# Autodesk Inventor assembly: 20263829
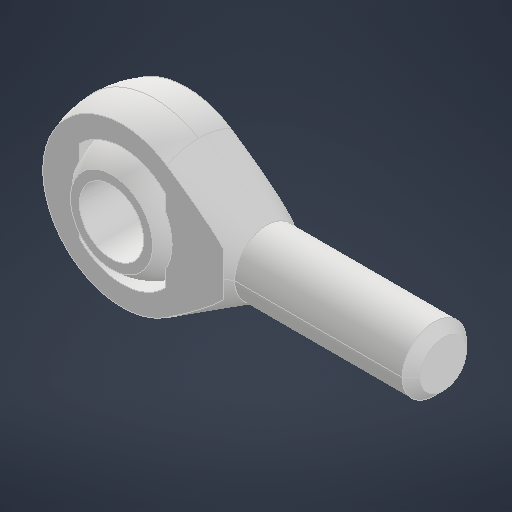
[picture p0: Inventor's stored thumbnail of the model, 512x512]
Saved by Autodesk Inventor 2026.1 (Build 301233000, 233)
## iProperties
Company: TraceParts S.A.
Created: 2026-06-12
Part Number: 20263829
Checked By: TraceParts S.A.
Catalog Web Link: www.traceparts.com
Document SubType Name: Assembly
Designer: TraceParts
Sending System: TraceParts v2
Major Version: 6.0
Minor Version: 0.0
Format Version: 0.0
Product Id: TraceParts v2
REFERENCE: 20263829
SUPPLIER: Essentra Components
DESIGN: Heavy Duty Rod End 12.0 54.0 M12 Steel
TraceParts.PartNumber: 90-24072024-043323
TraceParts.PartTitle: Heavy Duty Rod End 12.0 54.0 M12 Steel
TraceParts.InstanceId: 90-24072024-04332395OX6XW0EVGZUOK7QRY6KRUYN
TRACEPARTS: TRACEPARTS
TraceParts.PartLanguage: en
TraceParts.PartVersion: 1.0.1
Author: TraceParts
## Documents named in this file (4)
- C:\Users\share\OneDrive\Documents\Personal Projects\GOGO Kart\CAD\GOGO_KART_FSAE\Suspension\Suspension Parts\Front Upper Arm\Rod End CAD Files\185237224-9-20263829\20263829.iam
- C:\Users\share\OneDrive\Documents\Personal Projects\GOGO Kart\CAD\GOGO_KART_FSAE\Suspension\Suspension Parts\Front Upper Arm\Rod End CAD Files\185237224-9-20263829\20263829_01.ipt
- C:\Users\share\OneDrive\Documents\Personal Projects\GOGO Kart\CAD\GOGO_KART_FSAE\Suspension\Suspension Parts\Front Upper Arm\Rod End CAD Files\185237224-9-20263829\20263829_02.ipt
- C:\Users\share\OneDrive\Documents\Personal Projects\GOGO Kart\CAD\GOGO_KART_FSAE\Suspension\Suspension Parts\Front Upper Arm\Rod End CAD Files\185237224-9-20263829\20263829_03.ipt
## Components (3 placed, 3 different names)
1. 20263829_Temp_1:1
2. 20263829_Temp_2:1
3. 20263829_Temp_3:1
## Relationships (3: Mate 3)
- Mate:1
- Mate:2
- Mate:3
